# Autodesk Inventor assembly: SansRotor
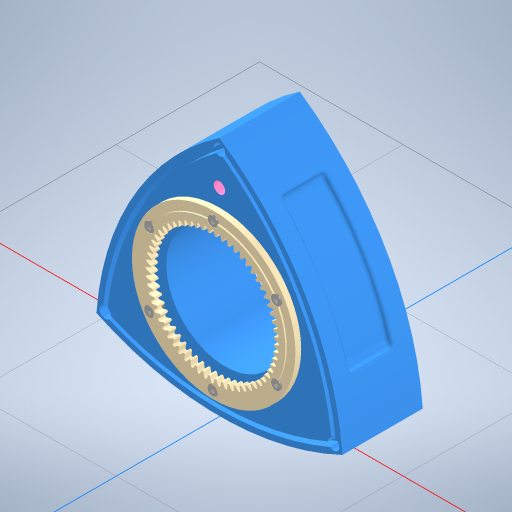
[picture p0: Inventor's stored thumbnail of the model, 512x512]
Saved by Autodesk Inventor 2024 (Build 280153000, 153)
## iProperties
Created: 2024-05-18
Part Number: SansRotor
Document SubType Name: Assembly
Designer: alexa
Author: alexa
## Documents named in this file (4)
- C:\Users\alexa\OneDrive\Documents\ANUL I\SEM 2\CAD\Tituleasa Ioana\SansRotor.iam
- C:\Users\alexa\OneDrive\Documents\ANUL I\SEM 2\CAD\Fisiere auxiliare teme Inventor\Fisiere auxiliare teme Inventor\7 - Wankel\Rotor.ipt
- C:\Users\alexa\OneDrive\Documents\ANUL I\SEM 2\CAD\Fisiere auxiliare teme Inventor\Fisiere auxiliare teme Inventor\7 - Wankel\Roata.ipt
- C:\Users\alexa\OneDrive\Documents\ANUL I\SEM 2\CAD\Tituleasa Ioana\SubAnsa-M4.iam
## Components (3 placed, 3 different names)
1. Rotor:1 — Mate:1, Mate:2, Mate:3, Mate:4, Mate:5
2. Roata:1 — Mate:4, Mate:5, Angle:1
3. SubAnsa-M4:1 [sub-assembly]
## Relationships (9: Mate 7, Angle 1, Insert 1)
- Mate:1: Rotor:1
- Mate:2: Rotor:1
- Mate:3: Rotor:1
- Mate:4: Rotor:1 ↔ Roata:1
- Mate:5: Rotor:1 ↔ Roata:1
- Angle:1 (0 deg): Roata:1
- [Mate]: Roata:1 ↔ SubAnsa-M4:1
- [Mate]: Roata:1 ↔ SubAnsa-M4:1
- [Insert]: Roata:1 ↔ SubAnsa-M4:1
